# Autodesk Inventor assembly: P1704_E1
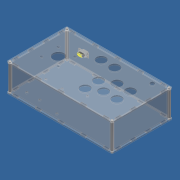
[picture p0: Inventor's stored thumbnail of the model, 180x180]
Saved by Autodesk Inventor 2015 SP2 (Build 190223200, 223)
## iProperties
Created: 2018-05-07
Part Number: P1704_E1
Project: Manette arcade
Description: Manette
Document SubType Name: Assembly
Designer: Alexandre.PICOTTE
Author: Alexandre.PICOTTE
## Documents named in this file (9)
- C:\Users\Alexandre.PICOTTE\Documents\P1704_Manettes\06_Dessins\Manette_arcade\P1704_E1.iam
- C:\Users\Alexandre.PICOTTE\Documents\P1704_Manettes\06_Dessins\Manette_arcade\P1704_006.ipt
- C:\Users\Alexandre.PICOTTE\Documents\P1704_Manettes\06_Dessins\Manette_arcade\P1704_005.ipt
- C:\Users\Alexandre.PICOTTE\Documents\P1704_Manettes\06_Dessins\Manette_arcade\P1704_003.ipt
- C:\Users\Alexandre.PICOTTE\Documents\P1704_Manettes\06_Dessins\Manette_arcade\P1704_004.ipt
- C:\Users\Alexandre.PICOTTE\Documents\P1704_Manettes\06_Dessins\Manette_arcade\P1704_002.ipt
- C:\Users\Alexandre.PICOTTE\Documents\Inventor\Content Center Files\R2015\fr-FR\D-Sub Male Crimp\D-Sub Male Crimp 9CKT.ipt
- C:\Users\Alexandre.PICOTTE\Documents\P1704_Manettes\06_Dessins\Manette_arcade\P1704_001_picotte_alexandre.ipt
- C:\Users\Alexandre.PICOTTE\Documents\Inventor\Content Center Files\R2015\fr-FR\ISO 4762(2)\ISO 4762 - M3 x 5ISO.ipt
## Components (19 placed, 8 different names)
1. P1704_006:1 — Affleurement:1, Placage:1, Placage:2, Affleurement:2, Placage:3, Placage:4, Placage:5, Placage:6, Placage:7, Placage:8, Placage:9, Placage:10, Logement:9, Logement:10, Logement:11, Logement:12
2. P1704_005:1 — Affleurement:1, Placage:1, Placage:2, Placage:12, Placage:13
3. P1704_005:2 — Affleurement:2, Placage:3, Placage:4
4. P1704_003:1 — Placage:5, Placage:6, Placage:7, Placage:11
5. P1704_004:1 — Placage:8, Placage:9, Placage:10, Placage:16, Placage:17
6. P1704_002:1 — Placage:11, Placage:12, Placage:13, Logement:1, Logement:2, Logement:3, Logement:4, Logement:5, Logement:6, Logement:7, Logement:8, Angle:2
7. Sertissage mâle D-Sub D-Sub Male Crimp 9CKT:1 — Placage:16, Placage:17, Angle:2
8. P1704_001_picotte_alexandre:1 — Logement:2
9. P1704_001_picotte_alexandre:2 — Logement:4
10. P1704_001_picotte_alexandre:3 — Logement:1
11. P1704_001_picotte_alexandre:4 — Logement:3
12. ISO 4762 M3 x 5:1 — Logement:5
13. ISO 4762 M3 x 5:2 — Logement:6
14. ISO 4762 M3 x 5:3 — Logement:7
15. ISO 4762 M3 x 5:4 — Logement:8
16. ISO 4762 M3 x 5:5 — Logement:9
17. ISO 4762 M3 x 5:6 — Logement:10
18. ISO 4762 M3 x 5:7 — Logement:11
19. ISO 4762 M3 x 5:8 — Logement:12
## Relationships (30: Mate 15, Insert 12, Flush 2, Angle 1)
- Affleurement:1 [Flush]: P1704_006:1 ↔ P1704_005:1
- Placage:1 [Mate]: P1704_006:1 ↔ P1704_005:1
- Placage:2 [Mate]: P1704_006:1 ↔ P1704_005:1
- Affleurement:2 [Flush]: P1704_006:1 ↔ P1704_005:2
- Placage:3 [Mate]: P1704_006:1 ↔ P1704_005:2
- Placage:4 [Mate]: P1704_006:1 ↔ P1704_005:2
- Placage:5 [Mate]: P1704_006:1 ↔ P1704_003:1
- Placage:6 [Mate]: P1704_006:1 ↔ P1704_003:1
- Placage:7 [Mate]: P1704_006:1 ↔ P1704_003:1
- Placage:8 [Mate]: P1704_006:1 ↔ P1704_004:1
- Placage:9 [Mate]: P1704_006:1 ↔ P1704_004:1
- Placage:10 [Mate]: P1704_006:1 ↔ P1704_004:1
- Placage:11 [Mate]: P1704_003:1 ↔ P1704_002:1
- Placage:12 [Mate]: P1704_005:1 ↔ P1704_002:1
- Placage:13 [Mate]: P1704_005:1 ↔ P1704_002:1
- Placage:16 [Mate]: P1704_004:1 ↔ Sertissage mâle D-Sub D-Sub Male Crimp 9CKT:1
- Placage:17 [Mate]: P1704_004:1 ↔ Sertissage mâle D-Sub D-Sub Male Crimp 9CKT:1
- Logement:1 [Insert]: P1704_002:1 ↔ P1704_001_picotte_alexandre:3
- Logement:2 [Insert]: P1704_002:1 ↔ P1704_001_picotte_alexandre:1
- Logement:3 [Insert]: P1704_002:1 ↔ P1704_001_picotte_alexandre:4
- Logement:4 [Insert]: P1704_002:1 ↔ P1704_001_picotte_alexandre:2
- Logement:5 [Insert]: P1704_002:1 ↔ ISO 4762 M3 x 5:1
- Logement:6 [Insert]: P1704_002:1 ↔ ISO 4762 M3 x 5:2
- Logement:7 [Insert]: P1704_002:1 ↔ ISO 4762 M3 x 5:3
- Logement:8 [Insert]: P1704_002:1 ↔ ISO 4762 M3 x 5:4
- Logement:9 [Insert]: P1704_006:1 ↔ ISO 4762 M3 x 5:5
- Logement:10 [Insert]: P1704_006:1 ↔ ISO 4762 M3 x 5:6
- Logement:11 [Insert]: P1704_006:1 ↔ ISO 4762 M3 x 5:7
- Logement:12 [Insert]: P1704_006:1 ↔ ISO 4762 M3 x 5:8
- Angle:2 (0 deg): P1704_002:1 ↔ Sertissage mâle D-Sub D-Sub Male Crimp 9CKT:1
